# Autodesk Inventor assembly: COM
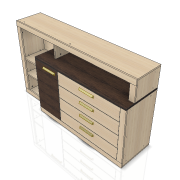
[picture p0: Inventor's stored thumbnail of the model, 180x180]
Saved by Autodesk Inventor 2024.3 (Build 283343000, 343)
## iProperties
Created: 2019-02-28
Document SubType Name: Assembly
Designer: SauliusD
Description: Commode
Part Number: COM
Author: SauliusD
## Documents named in this file (39)
- C:\W4INV 2024 Design\PROJECTS\Samples\Commode\COM.iam
- C:\W4INV 2024 Design\PROJECTS\Samples\Commode\COM_23.ipt
- C:\W4INV 2024 Design\PROJECTS\Samples\Commode\COM_10.ipt
- C:\W4INV 2024 Design\PROJECTS\Samples\Commode\COM_02.ipt
- C:\W4INV 2024 Design\PROJECTS\Samples\Commode\COM_16.ipt
- C:\W4INV 2024 Design\PROJECTS\Samples\Commode\COM_24.ipt
- C:\W4INV 2024 Design\PROJECTS\Samples\Commode\COM_11.ipt
- C:\W4INV 2024 Design\PROJECTS\Samples\Commode\COM_03.ipt
- C:\W4INV 2024 Design\PROJECTS\Samples\Commode\COM_17.ipt
- C:\W4INV 2024 Design\PROJECTS\Samples\Commode\COM_12.ipt
- C:\W4INV 2024 Design\PROJECTS\Samples\Commode\COM_25.ipt
- C:\W4INV 2024 Design\PROJECTS\Samples\Commode\COM_08.ipt
- C:\W4INV 2024 Design\PROJECTS\Samples\Commode\COM_04.ipt
- C:\W4INV 2024 Design\PROJECTS\Samples\Commode\COM_13.ipt
- C:\W4INV 2024 Design\PROJECTS\Samples\Commode\COM_05.ipt
- C:\W4INV 2024 Design\PROJECTS\Samples\Commode\COM_14.ipt
- C:\W4INV 2024 Design\PROJECTS\Samples\Commode\COM_18.ipt
- C:\W4INV 2024 Design\PROJECTS\Samples\Commode\COM_06.ipt
- C:\W4INV 2024 Design\PROJECTS\Samples\Commode\COM_07.ipt
- C:\W4INV 2024 Design\PROJECTS\Samples\Commode\COM_21.ipt
- C:\W4INV 2024 Design\PROJECTS\Samples\Commode\COM_20.ipt
- C:\W4INV 2024 Design\PROJECTS\Samples\Commode\COM_26.ipt
- C:\W4INV 2024 Design\PROJECTS\Samples\Commode\COM_19.ipt
- C:\W4INV 2024 Design\PROJECTS\Samples\Commode\COM_09.ipt
- C:\W4INV 2024 Design\PROJECTS\Samples\Commode\COM_15.ipt
- C:\W4INV 2024 Design\PROJECTS\Samples\Commode\SKL_COM_22.ipt
- C:\W4INV 2024 Design\PROJECTS\Samples\Commode\CommodePartial Pull Drawer 30 kg1\COM_01.iam
- C:\W4INV 2024 Design\_LIBRARY\Fixed joints\Minifix joint\MINIFIX D15 v2\Minifix D15 & Dowel L34 & Cap D15 PB T18 LH.ipt
- C:\W4INV 2024 Design\_LIBRARY\Holders\Shelf holder D5\Shelf support D5 L16 with hole covers.ipt
- C:\W4INV 2024 Design\_LIBRARY\Fixed joints\Dowel\DOWEL V2\Dowel 8x30 PB T=18.ipt
- C:\W4INV 2024 Design\_LIBRARY\Hinges\CONCEALED HINGE\Full Overlay Hinge Wood Screw Cup Wood Screw T18.iam
- C:\W4INV 2024 Design\_LIBRARY\Fixed joints\Minifix joint\MINIFIX D15 v2\Minifix D15 & Dowel L34 & Cap D15 PB T18 RH.ipt
- C:\W4INV 2024 Design\_LIBRARY\Fixed joints\Minifix joint\MINIFIX D15 v2\Minifix D15 & Dowel L34 & Cap D15 PB T18 BT.ipt
- C:\W4INV 2024 Design\PROJECTS\Samples\Commode\COM.iam Smart Hardware\ESTAMP Post 683110\ESTAMP Post 683110.iam
- C:\W4INV 2024 Design\PROJECTS\Samples\Commode\COM.iam Smart Hardware\ESTAMP Post 683111\ESTAMP Post 683111.iam
- C:\W4INV 2024 Design\LIBRARY\Fixed joints\Minifix joint\MINIFIX D15 v2.ipt
- C:\W4INV 2024 Design\LIBRARY\Holders\Shelf holder D5.ipt
- C:\W4INV 2024 Design\LIBRARY\Fixed joints\Dowel\DOWEL V2.ipt
- C:\W4INV 2024 Design\LIBRARY\Hinges\CONCEALED HINGE.iam
## Components (110 placed, 33 different names)
1. COM_23:1 — Axis Plane:1, Nestled Board Plane:1, Axis Plane:2, Nestled Board Plane:2, Axis Plane:3, Nestled Board Plane:3, Axis Plane:4, Nestled Board Plane:4, Axis Plane:5, Nestled Board Plane:5, Axis Plane:6, Nestled Board Plane:6, Axis Plane:7, Axis Plane:8, Axis Plane:9, Axis Plane:10, Axis Plane:11, Axis Plane:12, Axis Plane:29, Axis Plane:30, Axis Plane:31, Axis Plane:32, Axis Plane:33, Axis Plane:34, Axis Plane:35, Axis Plane:36, Pillar Board Side Plane :29, Pillar Board Side Plane :30, Pillar Board Side Plane :31, Axis Plane:69, Axis Plane:70
2. COM_10:1 — Pillar Board Side Plane :1, Pillar Board Side Plane :4, Pillar Board Side Plane :11, Pillar Board Side Plane :12, Side Board Plane:1, Side Board Plane:3, Side Board Plane:5, Side Board Plane:7, Pillar Board Side Plane :32, Pillar Board Side Plane :33, Pillar Board Side Plane :34
3. COM_02:1 — Nestled Board Plane:11, Nestled Board Plane:12, Pillar Board Side Plane :35, Pillar Board Side Plane :36, Pillar Board Side Plane :43, Pillar Board Side Plane :44
4. COM_16:1 — Pillar Board Side Plane :3, Pillar Board Side Plane :6, Pillar Board Side Plane :8, Pillar Board Side Plane :10
5. COM_24:1 — Nestled Board Plane:7, Nestled Board Plane:8, Nestled Board Plane:9, Nestled Board Plane:10, Axis Plane:13, Nestled Board Plane:13, Axis Plane:14, Axis Plane:15, Nestled Board Plane:15, Axis Plane:16, Axis Plane:17, Nestled Board Plane:17, Axis Plane:18, Axis Plane:19, Nestled Board Plane:19, Axis Plane:20, Axis Plane:21, Nestled Board Plane:21, Axis Plane:22, Axis Plane:23, Nestled Board Plane:23, Axis Plane:24, Axis Plane:25, Axis Plane:26, Axis Plane:27, Nestled Board Plane:27, Axis Plane:28, Nestled Board Plane:28, Axis Plane:37, Axis Plane:38, Axis Plane:39, Axis Plane:40, Axis Plane:41, Axis Plane:42, Axis Plane:43, Axis Plane:44, Nestled Board Plane:51, Nestled Board Plane:52
6. COM_11:1 — Pillar Board Side Plane :13, Pillar Board Side Plane :14, Pillar Board Side Plane :19, Pillar Board Side Plane :20, Side Board Plane:2, Side Board Plane:4, Side Board Plane:6, Side Board Plane:8, Side Board Plane:9, Side Board Plane:11, Side Board Plane:13, Side Board Plane:15, Cabinet Body Front  Edge Planar Face:1, Cabinet body Side Planar Face:1, Cabinet Body Front  Edge Planar Face:2, Cabinet body Side Planar Face:2, Nestled Board Plane:53, Nestled Board Plane:54
7. COM_03:1 — Nestled Board Plane:14, Nestled Board Plane:16, Nestled Board Plane:18, Nestled Board Plane:20, Nestled Board Plane:22, Nestled Board Plane:24, Nestled Board Plane:25, Nestled Board Plane:26, Pillar Board Side Plane :37, Pillar Board Side Plane :38, Pillar Board Side Plane :39
8. COM_17:1 — Pillar Board Side Plane :25, Pillar Board Side Plane :26, Pillar Board Side Plane :27, Pillar Board Side Plane :28, Pillar Board Side Plane :40, Pillar Board Side Plane :41, Pillar Board Side Plane :42
9. COM_12:1 — Pillar Board Side Plane :15, Pillar Board Side Plane :16, Pillar Board Side Plane :21, Pillar Board Side Plane :22, Side Board Plane:10, Side Board Plane:12, Side Board Plane:14, Side Board Plane:16
10. COM_25:1 — Axis Plane:45, Nestled Board Plane:29, Axis Plane:46, Nestled Board Plane:30, Axis Plane:47, Nestled Board Plane:31, Nestled Board Plane:43, Nestled Board Plane:44, Nestled Board Plane:45, Nestled Board Plane:46, Nestled Board Plane:49, Nestled Board Plane:50
11. COM_08:1 — Axis Plane:48, Nestled Board Plane:32, Axis Plane:49, Nestled Board Plane:33, Axis Plane:50, Nestled Board Plane:34, Axis Plane:59, Pillar Board Plane:1, Axis Plane:60, Pillar Board Plane:2, Pillar Board Plane:3, Pillar Board Plane:4, Axis Plane:63, Pillar Board Plane:5, Axis Plane:64, Pillar Board Plane:6
12. COM_04:1 — Axis Plane:51, Nestled Board Plane:35, Axis Plane:52, Nestled Board Plane:36, Nestled Board Plane:47, Nestled Board Plane:48
13. COM_13:1 — Axis Plane:61, Axis Plane:62, Axis Plane:65, Pillar Board Plane:7, Axis Plane:66, Pillar Board Plane:8, Axis Plane:67, Pillar Board Plane:9, Axis Plane:68, Pillar Board Plane:10
14. COM_05:1 — Axis Plane:53, Nestled Board Plane:37, Axis Plane:54, Nestled Board Plane:38, Axis Plane:55, Nestled Board Plane:39
15. COM_14:1 — Axis Plane:56, Nestled Board Plane:40, Axis Plane:57, Nestled Board Plane:41, Axis Plane:58, Nestled Board Plane:42
16. COM_18:1 — Pillar Board Side Plane :17, Pillar Board Side Plane :18, Pillar Board Side Plane :23, Pillar Board Side Plane :24
17. COM_06:1 — Flush:46, Flush:47
18. COM_21:1 — Top of drawer Box:1, Front of drawer Box:1, Right of drawer Box:1
19. COM_26:1 — Pillar Board Side Plane :2, Pillar Board Side Plane :5, Pillar Board Side Plane :7, Pillar Board Side Plane :9
20. COM_09:1
21. COM_15:1
22. Minifix D15 & Dowel L34 & Cap D15 PB T18 LH:2 — Axis Plane:1, Pillar Board Side Plane :1, Nestled Board Plane:1
23. Minifix D15 & Dowel L34 & Cap D15 PB T18 LH:3 — Axis Plane:2, Pillar Board Side Plane :2, Nestled Board Plane:2
24. Minifix D15 & Dowel L34 & Cap D15 PB T18 RH:4 — Axis Plane:3, Pillar Board Side Plane :3, Nestled Board Plane:3
25. Minifix D15 & Dowel L34 & Cap D15 PB T18 RH:5 — Axis Plane:4, Pillar Board Side Plane :4, Nestled Board Plane:4
26. Minifix D15 & Dowel L34 & Cap D15 PB T18 RH:6 — Axis Plane:5, Pillar Board Side Plane :5, Nestled Board Plane:5
27. Minifix D15 & Dowel L34 & Cap D15 PB T18 LH:7 — Axis Plane:6, Pillar Board Side Plane :6, Nestled Board Plane:6
28. Minifix D15 & Dowel L34 & Cap D15 PB T18 LH:8 — Axis Plane:7, Pillar Board Side Plane :7, Nestled Board Plane:7
29. Minifix D15 & Dowel L34 & Cap D15 PB T18 RH:9 — Axis Plane:8, Pillar Board Side Plane :8, Nestled Board Plane:8
30. Minifix D15 & Dowel L34 & Cap D15 PB T18 RH:10 — Axis Plane:9, Pillar Board Side Plane :9, Nestled Board Plane:9
31. Minifix D15 & Dowel L34 & Cap D15 PB T18 LH:11 — Axis Plane:10, Pillar Board Side Plane :10, Nestled Board Plane:10
32. Minifix D15 & Dowel L34 & Cap D15 PB T18 RH:12 — Axis Plane:11, Nestled Board Plane:11, Pillar Board Side Plane :11
33. Minifix D15 & Dowel L34 & Cap D15 PB T18 LH:13 — Axis Plane:12, Nestled Board Plane:12, Pillar Board Side Plane :12
34. Minifix D15 & Dowel L34 & Cap D15 PB T18 LH:14 — Axis Plane:13, Pillar Board Side Plane :13, Nestled Board Plane:13
35. Minifix D15 & Dowel L34 & Cap D15 PB T18 RH:15 — Axis Plane:14, Pillar Board Side Plane :14, Nestled Board Plane:14
36. Minifix D15 & Dowel L34 & Cap D15 PB T18 LH:16 — Axis Plane:15, Pillar Board Side Plane :15, Nestled Board Plane:15
37. Minifix D15 & Dowel L34 & Cap D15 PB T18 LH:17 — Axis Plane:16, Pillar Board Side Plane :16, Nestled Board Plane:16
38. Minifix D15 & Dowel L34 & Cap D15 PB T18 RH:18 — Axis Plane:17, Pillar Board Side Plane :17, Nestled Board Plane:17
39. Minifix D15 & Dowel L34 & Cap D15 PB T18 LH:19 — Axis Plane:18, Pillar Board Side Plane :18, Nestled Board Plane:18
40. Minifix D15 & Dowel L34 & Cap D15 PB T18 LH:20 — Axis Plane:19, Pillar Board Side Plane :19, Nestled Board Plane:19
41. Minifix D15 & Dowel L34 & Cap D15 PB T18 LH:21 — Axis Plane:20, Pillar Board Side Plane :20, Nestled Board Plane:20
42. Minifix D15 & Dowel L34 & Cap D15 PB T18 RH:22 — Axis Plane:21, Pillar Board Side Plane :21, Nestled Board Plane:21
43. Minifix D15 & Dowel L34 & Cap D15 PB T18 LH:23 — Axis Plane:22, Pillar Board Side Plane :22, Nestled Board Plane:22
44. Minifix D15 & Dowel L34 & Cap D15 PB T18 LH:24 — Axis Plane:23, Pillar Board Side Plane :23, Nestled Board Plane:23
45. Minifix D15 & Dowel L34 & Cap D15 PB T18 RH:25 — Axis Plane:24, Pillar Board Side Plane :24, Nestled Board Plane:24
46. Minifix D15 & Dowel L34 & Cap D15 PB T18 LH:26 — Axis Plane:25, Nestled Board Plane:25, Pillar Board Side Plane :25
47. Minifix D15 & Dowel L34 & Cap D15 PB T18 RH:27 — Axis Plane:26, Nestled Board Plane:26, Pillar Board Side Plane :26
48. Minifix D15 & Dowel L34 & Cap D15 PB T18 LH:28 — Axis Plane:27, Nestled Board Plane:27, Pillar Board Side Plane :27
49. Minifix D15 & Dowel L34 & Cap D15 PB T18 LH:29 — Axis Plane:28, Nestled Board Plane:28, Pillar Board Side Plane :28
50. Shelf support D5 L16 with hole covers:1 — Axis Plane:29, Shelf Pottom Plane:1, Side Board Plane:1
51. Shelf support D5 L16 with hole covers:2 — Axis Plane:30, Shelf Pottom Plane:2, Side Board Plane:2
52. Shelf support D5 L16 with hole covers:3 — Axis Plane:31, Shelf Pottom Plane:3, Side Board Plane:3
53. Shelf support D5 L16 with hole covers:4 — Axis Plane:32, Shelf Pottom Plane:4, Side Board Plane:4
54. Shelf support D5 L16 with hole covers:5 — Axis Plane:33, Shelf Pottom Plane:5, Side Board Plane:5
55. Shelf support D5 L16 with hole covers:6 — Axis Plane:34, Shelf Pottom Plane:6, Side Board Plane:6
56. Shelf support D5 L16 with hole covers:7 — Axis Plane:35, Shelf Pottom Plane:7, Side Board Plane:7
57. Shelf support D5 L16 with hole covers:8 — Axis Plane:36, Shelf Pottom Plane:8, Side Board Plane:8
58. Shelf support D5 L16 with hole covers:9 — Axis Plane:37, Shelf Pottom Plane:9, Side Board Plane:9
59. Shelf support D5 L16 with hole covers:10 — Axis Plane:38, Shelf Pottom Plane:10, Side Board Plane:10
60. Shelf support D5 L16 with hole covers:11 — Axis Plane:39, Shelf Pottom Plane:11, Side Board Plane:11
61. Shelf support D5 L16 with hole covers:12 — Axis Plane:40, Shelf Pottom Plane:12, Side Board Plane:12
62. Shelf support D5 L16 with hole covers:13 — Axis Plane:41, Shelf Pottom Plane:13, Side Board Plane:13
63. Shelf support D5 L16 with hole covers:14 — Axis Plane:42, Shelf Pottom Plane:14, Side Board Plane:14
64. Shelf support D5 L16 with hole covers:15 — Axis Plane:43, Shelf Pottom Plane:15, Side Board Plane:15
65. Shelf support D5 L16 with hole covers:16 — Axis Plane:44, Shelf Pottom Plane:16, Side Board Plane:16
66. Minifix D15 & Dowel L34 & Cap D15 PB T18 LH:30 — Axis Plane:45, Nestled Board Plane:29, Pillar Board Side Plane :29
67. Minifix D15 & Dowel L34 & Cap D15 PB T18 BT:31 — Axis Plane:46, Nestled Board Plane:30, Pillar Board Side Plane :30
68. Minifix D15 & Dowel L34 & Cap D15 PB T18 LH:32 — Axis Plane:47, Nestled Board Plane:31, Pillar Board Side Plane :31
69. Minifix D15 & Dowel L34 & Cap D15 PB T18 RH:33 — Axis Plane:48, Nestled Board Plane:32, Pillar Board Side Plane :32
70. Minifix D15 & Dowel L34 & Cap D15 PB T18 BT:34 — Axis Plane:49, Nestled Board Plane:33, Pillar Board Side Plane :33
71. Minifix D15 & Dowel L34 & Cap D15 PB T18 LH:35 — Axis Plane:50, Nestled Board Plane:34, Pillar Board Side Plane :34
72. Minifix D15 & Dowel L34 & Cap D15 PB T18 RH:36 — Axis Plane:51, Nestled Board Plane:35, Pillar Board Side Plane :35
73. Minifix D15 & Dowel L34 & Cap D15 PB T18 LH:37 — Axis Plane:52, Nestled Board Plane:36, Pillar Board Side Plane :36
74. Minifix D15 & Dowel L34 & Cap D15 PB T18 RH:38 — Axis Plane:53, Nestled Board Plane:37, Pillar Board Side Plane :37
75. Minifix D15 & Dowel L34 & Cap D15 PB T18 BT:39 — Axis Plane:54, Nestled Board Plane:38, Pillar Board Side Plane :38
76. Minifix D15 & Dowel L34 & Cap D15 PB T18 LH:40 — Axis Plane:55, Nestled Board Plane:39, Pillar Board Side Plane :39
77. Minifix D15 & Dowel L34 & Cap D15 PB T18 LH:41 — Axis Plane:56, Nestled Board Plane:40, Pillar Board Side Plane :40
78. Minifix D15 & Dowel L34 & Cap D15 PB T18 BT:42 — Axis Plane:57, Nestled Board Plane:41, Pillar Board Side Plane :41
79. Minifix D15 & Dowel L34 & Cap D15 PB T18 RH:43 — Axis Plane:58, Nestled Board Plane:42, Pillar Board Side Plane :42
80. Dowel 8x30 PB T=18:1 — Axis Plane:59, Nestled Board Plane:43, Pillar Board Plane:1
81. Dowel 8x30 PB T=18:2 — Axis Plane:60, Nestled Board Plane:44, Pillar Board Plane:2
82. Dowel 8x30 PB T=18:3 — Axis Plane:61, Nestled Board Plane:45, Pillar Board Plane:3
83. Dowel 8x30 PB T=18:4 — Axis Plane:62, Nestled Board Plane:46, Pillar Board Plane:4
84. Dowel 8x30 PB T=18:5 — Axis Plane:63, Nestled Board Plane:47, Pillar Board Plane:5
85. Dowel 8x30 PB T=18:6 — Axis Plane:64, Nestled Board Plane:48, Pillar Board Plane:6
86. Dowel 8x30 PB T=18:7 — Axis Plane:65, Nestled Board Plane:49, Pillar Board Plane:7
87. Dowel 8x30 PB T=18:8 — Axis Plane:66, Nestled Board Plane:50, Pillar Board Plane:8
88. Dowel 8x30 PB T=18:9 — Axis Plane:67, Nestled Board Plane:51, Pillar Board Plane:9
89. Dowel 8x30 PB T=18:10 — Axis Plane:68, Nestled Board Plane:52, Pillar Board Plane:10
90. Full Overlay Hinge Wood Screw Cup Wood Screw T18:1 [sub-assembly] — Hinge Center Axis Plane:1, Cabinet Body Front  Edge Planar Face:1, Cabinet body Side Planar Face:1
91. Full Overlay Hinge Wood Screw Cup Wood Screw T18:2 [sub-assembly] — Hinge Center Axis Plane:2, Cabinet Body Front  Edge Planar Face:2, Cabinet body Side Planar Face:2
92. Minifix D15 & Dowel L34 & Cap D15 PB T18 LH:45 — Axis Plane:69, Nestled Board Plane:53, Pillar Board Side Plane :43
93. Minifix D15 & Dowel L34 & Cap D15 PB T18 RH:46 — Axis Plane:70, Nestled Board Plane:54, Pillar Board Side Plane :44
94. ESTAMP Post 683111:1 [sub-assembly]
95. COM_07:1
96. ESTAMP Post 683110:1 [sub-assembly]
97. COM_07:2
98. ESTAMP Post 683110:2 [sub-assembly]
99. COM_07:3
100. ESTAMP Post 683110:3 [sub-assembly]
101. COM_07:4
102. ESTAMP Post 683110:4 [sub-assembly]
103. COM_20:1 — Shelf Pottom Plane:1, Shelf Pottom Plane:2, Shelf Pottom Plane:5, Shelf Pottom Plane:6
104. COM_20:2 — Shelf Pottom Plane:3, Shelf Pottom Plane:4, Shelf Pottom Plane:7, Shelf Pottom Plane:8
105. COM_19:1 — Shelf Pottom Plane:9, Shelf Pottom Plane:10, Shelf Pottom Plane:13, Shelf Pottom Plane:14
106. COM_19:2 — Shelf Pottom Plane:11, Shelf Pottom Plane:12, Shelf Pottom Plane:15, Shelf Pottom Plane:16
107. COM_01:1 [sub-assembly] — Top of drawer Box:1, Front of drawer Box:1, Right of drawer Box:1
108. COM_01:2 [sub-assembly]
109. COM_01:3 [sub-assembly]
110. COM_01:4 [sub-assembly]
## Component patterns: (4 elements, first: COM_07:1 + ESTAMP Post 683110:1), (2 elements, first: COM_20:1), (2 elements, first: COM_19:1), (4 elements, first: COM_01:1)
## Relationships (221: Mate 170, Flush 51)
- Top of drawer Box:1 [Flush]: COM_21:1 ↔ COM_01:1
- Front of drawer Box:1 [Flush]: COM_21:1 ↔ COM_01:1
- Right of drawer Box:1 [Flush]: COM_21:1 ↔ COM_01:1
- Axis Plane:1 [Mate]: COM_23:1 ↔ Minifix D15 & Dowel L34 & Cap D15 PB T18 LH:2
- Pillar Board Side Plane :1 [Flush] (18 mm): COM_10:1 ↔ Minifix D15 & Dowel L34 & Cap D15 PB T18 LH:2
- Nestled Board Plane:1 [Mate]: COM_23:1 ↔ Minifix D15 & Dowel L34 & Cap D15 PB T18 LH:2
- Axis Plane:2 [Mate]: COM_23:1 ↔ Minifix D15 & Dowel L34 & Cap D15 PB T18 LH:3
- Pillar Board Side Plane :2 [Flush] (18 mm): COM_26:1 ↔ Minifix D15 & Dowel L34 & Cap D15 PB T18 LH:3
- Nestled Board Plane:2 [Mate]: COM_23:1 ↔ Minifix D15 & Dowel L34 & Cap D15 PB T18 LH:3
- Axis Plane:3 [Mate]: COM_23:1 ↔ Minifix D15 & Dowel L34 & Cap D15 PB T18 RH:4
- Pillar Board Side Plane :3 [Flush] (18 mm): COM_16:1 ↔ Minifix D15 & Dowel L34 & Cap D15 PB T18 RH:4
- Nestled Board Plane:3 [Mate]: COM_23:1 ↔ Minifix D15 & Dowel L34 & Cap D15 PB T18 RH:4
- Axis Plane:4 [Mate]: COM_23:1 ↔ Minifix D15 & Dowel L34 & Cap D15 PB T18 RH:5
- Pillar Board Side Plane :4 [Flush] (18 mm): COM_10:1 ↔ Minifix D15 & Dowel L34 & Cap D15 PB T18 RH:5
- Nestled Board Plane:4 [Mate]: COM_23:1 ↔ Minifix D15 & Dowel L34 & Cap D15 PB T18 RH:5
- Axis Plane:5 [Mate]: COM_23:1 ↔ Minifix D15 & Dowel L34 & Cap D15 PB T18 RH:6
- Pillar Board Side Plane :5 [Flush] (18 mm): COM_26:1 ↔ Minifix D15 & Dowel L34 & Cap D15 PB T18 RH:6
- Nestled Board Plane:5 [Mate]: COM_23:1 ↔ Minifix D15 & Dowel L34 & Cap D15 PB T18 RH:6
- Axis Plane:6 [Mate]: COM_23:1 ↔ Minifix D15 & Dowel L34 & Cap D15 PB T18 LH:7
- Pillar Board Side Plane :6 [Flush] (18 mm): COM_16:1 ↔ Minifix D15 & Dowel L34 & Cap D15 PB T18 LH:7
- Nestled Board Plane:6 [Mate]: COM_23:1 ↔ Minifix D15 & Dowel L34 & Cap D15 PB T18 LH:7
- Axis Plane:7 [Mate]: COM_23:1 ↔ Minifix D15 & Dowel L34 & Cap D15 PB T18 LH:8
- Pillar Board Side Plane :7 [Flush] (18 mm): COM_26:1 ↔ Minifix D15 & Dowel L34 & Cap D15 PB T18 LH:8
- Nestled Board Plane:7 [Mate]: COM_24:1 ↔ Minifix D15 & Dowel L34 & Cap D15 PB T18 LH:8
- Axis Plane:8 [Mate]: COM_23:1 ↔ Minifix D15 & Dowel L34 & Cap D15 PB T18 RH:9
- Pillar Board Side Plane :8 [Flush] (18 mm): COM_16:1 ↔ Minifix D15 & Dowel L34 & Cap D15 PB T18 RH:9
- Nestled Board Plane:8 [Mate]: COM_24:1 ↔ Minifix D15 & Dowel L34 & Cap D15 PB T18 RH:9
- Axis Plane:9 [Mate]: COM_23:1 ↔ Minifix D15 & Dowel L34 & Cap D15 PB T18 RH:10
- Pillar Board Side Plane :9 [Flush] (18 mm): COM_26:1 ↔ Minifix D15 & Dowel L34 & Cap D15 PB T18 RH:10
- Nestled Board Plane:9 [Mate]: COM_24:1 ↔ Minifix D15 & Dowel L34 & Cap D15 PB T18 RH:10
- Axis Plane:10 [Mate]: COM_23:1 ↔ Minifix D15 & Dowel L34 & Cap D15 PB T18 LH:11
- Pillar Board Side Plane :10 [Flush] (18 mm): COM_16:1 ↔ Minifix D15 & Dowel L34 & Cap D15 PB T18 LH:11
- Nestled Board Plane:10 [Mate]: COM_24:1 ↔ Minifix D15 & Dowel L34 & Cap D15 PB T18 LH:11
- Axis Plane:11 [Mate]: COM_23:1 ↔ Minifix D15 & Dowel L34 & Cap D15 PB T18 RH:12
- Nestled Board Plane:11 [Mate]: COM_02:1 ↔ Minifix D15 & Dowel L34 & Cap D15 PB T18 RH:12
- Pillar Board Side Plane :11 [Flush] (18 mm): COM_10:1 ↔ Minifix D15 & Dowel L34 & Cap D15 PB T18 RH:12
- Axis Plane:12 [Mate]: COM_23:1 ↔ Minifix D15 & Dowel L34 & Cap D15 PB T18 LH:13
- Nestled Board Plane:12 [Mate]: COM_02:1 ↔ Minifix D15 & Dowel L34 & Cap D15 PB T18 LH:13
- Pillar Board Side Plane :12 [Flush] (18 mm): COM_10:1 ↔ Minifix D15 & Dowel L34 & Cap D15 PB T18 LH:13
- Axis Plane:13 [Mate]: COM_24:1 ↔ Minifix D15 & Dowel L34 & Cap D15 PB T18 LH:14
- Pillar Board Side Plane :13 [Flush] (18 mm): COM_11:1 ↔ Minifix D15 & Dowel L34 & Cap D15 PB T18 LH:14
- Nestled Board Plane:13 [Mate]: COM_24:1 ↔ Minifix D15 & Dowel L34 & Cap D15 PB T18 LH:14
- Axis Plane:14 [Mate]: COM_24:1 ↔ Minifix D15 & Dowel L34 & Cap D15 PB T18 RH:15
- Pillar Board Side Plane :14 [Flush] (18 mm): COM_11:1 ↔ Minifix D15 & Dowel L34 & Cap D15 PB T18 RH:15
- Nestled Board Plane:14 [Mate]: COM_03:1 ↔ Minifix D15 & Dowel L34 & Cap D15 PB T18 RH:15
- Axis Plane:15 [Mate]: COM_24:1 ↔ Minifix D15 & Dowel L34 & Cap D15 PB T18 LH:16
- Pillar Board Side Plane :15 [Flush] (18 mm): COM_12:1 ↔ Minifix D15 & Dowel L34 & Cap D15 PB T18 LH:16
- Nestled Board Plane:15 [Mate]: COM_24:1 ↔ Minifix D15 & Dowel L34 & Cap D15 PB T18 LH:16
- Axis Plane:16 [Mate]: COM_24:1 ↔ Minifix D15 & Dowel L34 & Cap D15 PB T18 LH:17
- Pillar Board Side Plane :16 [Flush] (18 mm): COM_12:1 ↔ Minifix D15 & Dowel L34 & Cap D15 PB T18 LH:17
- Nestled Board Plane:16 [Mate]: COM_03:1 ↔ Minifix D15 & Dowel L34 & Cap D15 PB T18 LH:17
- Axis Plane:17 [Mate]: COM_24:1 ↔ Minifix D15 & Dowel L34 & Cap D15 PB T18 RH:18
- Pillar Board Side Plane :17 [Flush] (18 mm): COM_18:1 ↔ Minifix D15 & Dowel L34 & Cap D15 PB T18 RH:18
- Nestled Board Plane:17 [Mate]: COM_24:1 ↔ Minifix D15 & Dowel L34 & Cap D15 PB T18 RH:18
- Axis Plane:18 [Mate]: COM_24:1 ↔ Minifix D15 & Dowel L34 & Cap D15 PB T18 LH:19
- Pillar Board Side Plane :18 [Flush] (18 mm): COM_18:1 ↔ Minifix D15 & Dowel L34 & Cap D15 PB T18 LH:19
- Nestled Board Plane:18 [Mate]: COM_03:1 ↔ Minifix D15 & Dowel L34 & Cap D15 PB T18 LH:19
- Axis Plane:19 [Mate]: COM_24:1 ↔ Minifix D15 & Dowel L34 & Cap D15 PB T18 LH:20
- Pillar Board Side Plane :19 [Flush] (18 mm): COM_11:1 ↔ Minifix D15 & Dowel L34 & Cap D15 PB T18 LH:20
- Nestled Board Plane:19 [Mate]: COM_24:1 ↔ Minifix D15 & Dowel L34 & Cap D15 PB T18 LH:20
- Axis Plane:20 [Mate]: COM_24:1 ↔ Minifix D15 & Dowel L34 & Cap D15 PB T18 LH:21
- Pillar Board Side Plane :20 [Flush] (18 mm): COM_11:1 ↔ Minifix D15 & Dowel L34 & Cap D15 PB T18 LH:21
- Nestled Board Plane:20 [Mate]: COM_03:1 ↔ Minifix D15 & Dowel L34 & Cap D15 PB T18 LH:21
- Axis Plane:21 [Mate]: COM_24:1 ↔ Minifix D15 & Dowel L34 & Cap D15 PB T18 RH:22
- Pillar Board Side Plane :21 [Flush] (18 mm): COM_12:1 ↔ Minifix D15 & Dowel L34 & Cap D15 PB T18 RH:22
- Nestled Board Plane:21 [Mate]: COM_24:1 ↔ Minifix D15 & Dowel L34 & Cap D15 PB T18 RH:22
- Axis Plane:22 [Mate]: COM_24:1 ↔ Minifix D15 & Dowel L34 & Cap D15 PB T18 LH:23
- Pillar Board Side Plane :22 [Flush] (18 mm): COM_12:1 ↔ Minifix D15 & Dowel L34 & Cap D15 PB T18 LH:23
- Nestled Board Plane:22 [Mate]: COM_03:1 ↔ Minifix D15 & Dowel L34 & Cap D15 PB T18 LH:23
- Axis Plane:23 [Mate]: COM_24:1 ↔ Minifix D15 & Dowel L34 & Cap D15 PB T18 LH:24
- Pillar Board Side Plane :23 [Flush] (18 mm): COM_18:1 ↔ Minifix D15 & Dowel L34 & Cap D15 PB T18 LH:24
- Nestled Board Plane:23 [Mate]: COM_24:1 ↔ Minifix D15 & Dowel L34 & Cap D15 PB T18 LH:24
- Axis Plane:24 [Mate]: COM_24:1 ↔ Minifix D15 & Dowel L34 & Cap D15 PB T18 RH:25
- Pillar Board Side Plane :24 [Flush] (18 mm): COM_18:1 ↔ Minifix D15 & Dowel L34 & Cap D15 PB T18 RH:25
- Nestled Board Plane:24 [Mate]: COM_03:1 ↔ Minifix D15 & Dowel L34 & Cap D15 PB T18 RH:25
- Axis Plane:25 [Mate]: COM_24:1 ↔ Minifix D15 & Dowel L34 & Cap D15 PB T18 LH:26
- Nestled Board Plane:25 [Mate]: COM_03:1 ↔ Minifix D15 & Dowel L34 & Cap D15 PB T18 LH:26
- Pillar Board Side Plane :25 [Flush] (18 mm): COM_17:1 ↔ Minifix D15 & Dowel L34 & Cap D15 PB T18 LH:26
- Axis Plane:26 [Mate]: COM_24:1 ↔ Minifix D15 & Dowel L34 & Cap D15 PB T18 RH:27
- Nestled Board Plane:26 [Mate]: COM_03:1 ↔ Minifix D15 & Dowel L34 & Cap D15 PB T18 RH:27
- Pillar Board Side Plane :26 [Flush] (18 mm): COM_17:1 ↔ Minifix D15 & Dowel L34 & Cap D15 PB T18 RH:27
- Axis Plane:27 [Mate]: COM_24:1 ↔ Minifix D15 & Dowel L34 & Cap D15 PB T18 LH:28
- Nestled Board Plane:27 [Mate]: COM_24:1 ↔ Minifix D15 & Dowel L34 & Cap D15 PB T18 LH:28
- Pillar Board Side Plane :27 [Flush] (18 mm): COM_17:1 ↔ Minifix D15 & Dowel L34 & Cap D15 PB T18 LH:28
- Axis Plane:28 [Mate]: COM_24:1 ↔ Minifix D15 & Dowel L34 & Cap D15 PB T18 LH:29
- Nestled Board Plane:28 [Mate]: COM_24:1 ↔ Minifix D15 & Dowel L34 & Cap D15 PB T18 LH:29
- Pillar Board Side Plane :28 [Flush] (18 mm): COM_17:1 ↔ Minifix D15 & Dowel L34 & Cap D15 PB T18 LH:29
- Axis Plane:29 [Mate]: COM_23:1 ↔ Shelf support D5 L16 with hole covers:1
- Shelf Pottom Plane:1 [Mate] (2.5 mm): Shelf support D5 L16 with hole covers:1 ↔ COM_20:1
- Side Board Plane:1 [Mate]: COM_10:1 ↔ Shelf support D5 L16 with hole covers:1
- Axis Plane:30 [Mate]: COM_23:1 ↔ Shelf support D5 L16 with hole covers:2
- Shelf Pottom Plane:2 [Mate] (2.5 mm): Shelf support D5 L16 with hole covers:2 ↔ COM_20:1
- Side Board Plane:2 [Mate]: COM_11:1 ↔ Shelf support D5 L16 with hole covers:2
- Axis Plane:31 [Mate]: COM_23:1 ↔ Shelf support D5 L16 with hole covers:3
- Shelf Pottom Plane:3 [Mate] (2.5 mm): Shelf support D5 L16 with hole covers:3 ↔ COM_20:2
- Side Board Plane:3 [Mate]: COM_10:1 ↔ Shelf support D5 L16 with hole covers:3
- Axis Plane:32 [Mate]: COM_23:1 ↔ Shelf support D5 L16 with hole covers:4
- Shelf Pottom Plane:4 [Mate] (2.5 mm): Shelf support D5 L16 with hole covers:4 ↔ COM_20:2
- Side Board Plane:4 [Mate]: COM_11:1 ↔ Shelf support D5 L16 with hole covers:4
- Axis Plane:33 [Mate]: COM_23:1 ↔ Shelf support D5 L16 with hole covers:5
- Shelf Pottom Plane:5 [Mate] (2.5 mm): Shelf support D5 L16 with hole covers:5 ↔ COM_20:1
- Side Board Plane:5 [Mate]: COM_10:1 ↔ Shelf support D5 L16 with hole covers:5
- Axis Plane:34 [Mate]: COM_23:1 ↔ Shelf support D5 L16 with hole covers:6
- Shelf Pottom Plane:6 [Mate] (2.5 mm): Shelf support D5 L16 with hole covers:6 ↔ COM_20:1
- Side Board Plane:6 [Mate]: COM_11:1 ↔ Shelf support D5 L16 with hole covers:6
- Axis Plane:35 [Mate]: COM_23:1 ↔ Shelf support D5 L16 with hole covers:7
- Shelf Pottom Plane:7 [Mate] (2.5 mm): Shelf support D5 L16 with hole covers:7 ↔ COM_20:2
- Side Board Plane:7 [Mate]: COM_10:1 ↔ Shelf support D5 L16 with hole covers:7
- Axis Plane:36 [Mate]: COM_23:1 ↔ Shelf support D5 L16 with hole covers:8
- Shelf Pottom Plane:8 [Mate] (2.5 mm): Shelf support D5 L16 with hole covers:8 ↔ COM_20:2
- Side Board Plane:8 [Mate]: COM_11:1 ↔ Shelf support D5 L16 with hole covers:8
- Axis Plane:37 [Mate]: COM_24:1 ↔ Shelf support D5 L16 with hole covers:9
- Shelf Pottom Plane:9 [Mate] (2.5 mm): Shelf support D5 L16 with hole covers:9 ↔ COM_19:1
- Side Board Plane:9 [Mate]: COM_11:1 ↔ Shelf support D5 L16 with hole covers:9
- Axis Plane:38 [Mate]: COM_24:1 ↔ Shelf support D5 L16 with hole covers:10
- Shelf Pottom Plane:10 [Mate] (2.5 mm): Shelf support D5 L16 with hole covers:10 ↔ COM_19:1
- Side Board Plane:10 [Mate]: COM_12:1 ↔ Shelf support D5 L16 with hole covers:10
- Axis Plane:39 [Mate]: COM_24:1 ↔ Shelf support D5 L16 with hole covers:11
- Shelf Pottom Plane:11 [Mate] (2.5 mm): Shelf support D5 L16 with hole covers:11 ↔ COM_19:2
- Side Board Plane:11 [Mate]: COM_11:1 ↔ Shelf support D5 L16 with hole covers:11
- Axis Plane:40 [Mate]: COM_24:1 ↔ Shelf support D5 L16 with hole covers:12
- Shelf Pottom Plane:12 [Mate] (2.5 mm): Shelf support D5 L16 with hole covers:12 ↔ COM_19:2
- Side Board Plane:12 [Mate]: COM_12:1 ↔ Shelf support D5 L16 with hole covers:12
- Axis Plane:41 [Mate]: COM_24:1 ↔ Shelf support D5 L16 with hole covers:13
- Shelf Pottom Plane:13 [Mate] (2.5 mm): Shelf support D5 L16 with hole covers:13 ↔ COM_19:1
- Side Board Plane:13 [Mate]: COM_11:1 ↔ Shelf support D5 L16 with hole covers:13
- Axis Plane:42 [Mate]: COM_24:1 ↔ Shelf support D5 L16 with hole covers:14
- Shelf Pottom Plane:14 [Mate] (2.5 mm): Shelf support D5 L16 with hole covers:14 ↔ COM_19:1
- Side Board Plane:14 [Mate]: COM_12:1 ↔ Shelf support D5 L16 with hole covers:14
- Axis Plane:43 [Mate]: COM_24:1 ↔ Shelf support D5 L16 with hole covers:15
- Shelf Pottom Plane:15 [Mate] (2.5 mm): Shelf support D5 L16 with hole covers:15 ↔ COM_19:2
- Side Board Plane:15 [Mate]: COM_11:1 ↔ Shelf support D5 L16 with hole covers:15
- Axis Plane:44 [Mate]: COM_24:1 ↔ Shelf support D5 L16 with hole covers:16
- Shelf Pottom Plane:16 [Mate] (2.5 mm): Shelf support D5 L16 with hole covers:16 ↔ COM_19:2
- Side Board Plane:16 [Mate]: COM_12:1 ↔ Shelf support D5 L16 with hole covers:16
- Axis Plane:45 [Mate]: COM_25:1 ↔ Minifix D15 & Dowel L34 & Cap D15 PB T18 LH:30
- Nestled Board Plane:29 [Mate]: COM_25:1 ↔ Minifix D15 & Dowel L34 & Cap D15 PB T18 LH:30
- Pillar Board Side Plane :29 [Flush] (18 mm): COM_23:1 ↔ Minifix D15 & Dowel L34 & Cap D15 PB T18 LH:30
- Axis Plane:46 [Mate]: COM_25:1 ↔ Minifix D15 & Dowel L34 & Cap D15 PB T18 BT:31
- Nestled Board Plane:30 [Mate]: COM_25:1 ↔ Minifix D15 & Dowel L34 & Cap D15 PB T18 BT:31
- Pillar Board Side Plane :30 [Flush] (18 mm): COM_23:1 ↔ Minifix D15 & Dowel L34 & Cap D15 PB T18 BT:31
- Axis Plane:47 [Mate]: COM_25:1 ↔ Minifix D15 & Dowel L34 & Cap D15 PB T18 LH:32
- Nestled Board Plane:31 [Mate]: COM_25:1 ↔ Minifix D15 & Dowel L34 & Cap D15 PB T18 LH:32
- Pillar Board Side Plane :31 [Flush] (18 mm): COM_23:1 ↔ Minifix D15 & Dowel L34 & Cap D15 PB T18 LH:32
- Axis Plane:48 [Mate]: COM_08:1 ↔ Minifix D15 & Dowel L34 & Cap D15 PB T18 RH:33
- Nestled Board Plane:32 [Mate]: COM_08:1 ↔ Minifix D15 & Dowel L34 & Cap D15 PB T18 RH:33
- Pillar Board Side Plane :32 [Flush] (18 mm): COM_10:1 ↔ Minifix D15 & Dowel L34 & Cap D15 PB T18 RH:33
- Axis Plane:49 [Mate]: COM_08:1 ↔ Minifix D15 & Dowel L34 & Cap D15 PB T18 BT:34
- Nestled Board Plane:33 [Mate]: COM_08:1 ↔ Minifix D15 & Dowel L34 & Cap D15 PB T18 BT:34
- Pillar Board Side Plane :33 [Flush] (18 mm): COM_10:1 ↔ Minifix D15 & Dowel L34 & Cap D15 PB T18 BT:34
- Axis Plane:50 [Mate]: COM_08:1 ↔ Minifix D15 & Dowel L34 & Cap D15 PB T18 LH:35
- Nestled Board Plane:34 [Mate]: COM_08:1 ↔ Minifix D15 & Dowel L34 & Cap D15 PB T18 LH:35
- Pillar Board Side Plane :34 [Flush] (18 mm): COM_10:1 ↔ Minifix D15 & Dowel L34 & Cap D15 PB T18 LH:35
- Axis Plane:51 [Mate]: COM_04:1 ↔ Minifix D15 & Dowel L34 & Cap D15 PB T18 RH:36
- Nestled Board Plane:35 [Mate]: COM_04:1 ↔ Minifix D15 & Dowel L34 & Cap D15 PB T18 RH:36
- Pillar Board Side Plane :35 [Flush] (18 mm): COM_02:1 ↔ Minifix D15 & Dowel L34 & Cap D15 PB T18 RH:36
- Axis Plane:52 [Mate]: COM_04:1 ↔ Minifix D15 & Dowel L34 & Cap D15 PB T18 LH:37
- Nestled Board Plane:36 [Mate]: COM_04:1 ↔ Minifix D15 & Dowel L34 & Cap D15 PB T18 LH:37
- Pillar Board Side Plane :36 [Flush] (18 mm): COM_02:1 ↔ Minifix D15 & Dowel L34 & Cap D15 PB T18 LH:37
- Axis Plane:53 [Mate]: COM_05:1 ↔ Minifix D15 & Dowel L34 & Cap D15 PB T18 RH:38
- Nestled Board Plane:37 [Mate]: COM_05:1 ↔ Minifix D15 & Dowel L34 & Cap D15 PB T18 RH:38
- Pillar Board Side Plane :37 [Flush] (18 mm): COM_03:1 ↔ Minifix D15 & Dowel L34 & Cap D15 PB T18 RH:38
- Axis Plane:54 [Mate]: COM_05:1 ↔ Minifix D15 & Dowel L34 & Cap D15 PB T18 BT:39
- Nestled Board Plane:38 [Mate]: COM_05:1 ↔ Minifix D15 & Dowel L34 & Cap D15 PB T18 BT:39
- Pillar Board Side Plane :38 [Flush] (18 mm): COM_03:1 ↔ Minifix D15 & Dowel L34 & Cap D15 PB T18 BT:39
- Axis Plane:55 [Mate]: COM_05:1 ↔ Minifix D15 & Dowel L34 & Cap D15 PB T18 LH:40
- Nestled Board Plane:39 [Mate]: COM_05:1 ↔ Minifix D15 & Dowel L34 & Cap D15 PB T18 LH:40
- Pillar Board Side Plane :39 [Flush] (18 mm): COM_03:1 ↔ Minifix D15 & Dowel L34 & Cap D15 PB T18 LH:40
- Axis Plane:56 [Mate]: COM_14:1 ↔ Minifix D15 & Dowel L34 & Cap D15 PB T18 LH:41
- Nestled Board Plane:40 [Mate]: COM_14:1 ↔ Minifix D15 & Dowel L34 & Cap D15 PB T18 LH:41
- Pillar Board Side Plane :40 [Flush] (18 mm): COM_17:1 ↔ Minifix D15 & Dowel L34 & Cap D15 PB T18 LH:41
- Axis Plane:57 [Mate]: COM_14:1 ↔ Minifix D15 & Dowel L34 & Cap D15 PB T18 BT:42
- Nestled Board Plane:41 [Mate]: COM_14:1 ↔ Minifix D15 & Dowel L34 & Cap D15 PB T18 BT:42
- Pillar Board Side Plane :41 [Flush] (18 mm): COM_17:1 ↔ Minifix D15 & Dowel L34 & Cap D15 PB T18 BT:42
- Axis Plane:58 [Mate]: COM_14:1 ↔ Minifix D15 & Dowel L34 & Cap D15 PB T18 RH:43
- Nestled Board Plane:42 [Mate]: COM_14:1 ↔ Minifix D15 & Dowel L34 & Cap D15 PB T18 RH:43
- Pillar Board Side Plane :42 [Flush] (18 mm): COM_17:1 ↔ Minifix D15 & Dowel L34 & Cap D15 PB T18 RH:43
- Axis Plane:59 [Mate]: COM_08:1 ↔ Dowel 8x30 PB T=18:1
- Nestled Board Plane:43 [Mate]: COM_25:1 ↔ Dowel 8x30 PB T=18:1
- Pillar Board Plane:1 [Mate] (-9 mm): COM_08:1 ↔ Dowel 8x30 PB T=18:1
- Axis Plane:60 [Mate]: COM_08:1 ↔ Dowel 8x30 PB T=18:2
- Nestled Board Plane:44 [Mate]: COM_25:1 ↔ Dowel 8x30 PB T=18:2
- Pillar Board Plane:2 [Mate] (-9 mm): COM_08:1 ↔ Dowel 8x30 PB T=18:2
- Axis Plane:61 [Mate]: COM_13:1 ↔ Dowel 8x30 PB T=18:3
- Nestled Board Plane:45 [Mate]: COM_25:1 ↔ Dowel 8x30 PB T=18:3
- Pillar Board Plane:3 [Mate] (-9 mm): COM_08:1 ↔ Dowel 8x30 PB T=18:3
- Axis Plane:62 [Mate]: COM_13:1 ↔ Dowel 8x30 PB T=18:4
- Nestled Board Plane:46 [Mate]: COM_25:1 ↔ Dowel 8x30 PB T=18:4
- Pillar Board Plane:4 [Mate] (-9 mm): COM_08:1 ↔ Dowel 8x30 PB T=18:4
- Axis Plane:63 [Mate]: COM_08:1 ↔ Dowel 8x30 PB T=18:5
- Nestled Board Plane:47 [Mate]: COM_04:1 ↔ Dowel 8x30 PB T=18:5
- Pillar Board Plane:5 [Mate] (-9 mm): COM_08:1 ↔ Dowel 8x30 PB T=18:5
- Axis Plane:64 [Mate]: COM_08:1 ↔ Dowel 8x30 PB T=18:6
- Nestled Board Plane:48 [Mate]: COM_04:1 ↔ Dowel 8x30 PB T=18:6
- Pillar Board Plane:6 [Mate] (-9 mm): COM_08:1 ↔ Dowel 8x30 PB T=18:6
- Axis Plane:65 [Mate]: COM_13:1 ↔ Dowel 8x30 PB T=18:7
- Nestled Board Plane:49 [Mate]: COM_25:1 ↔ Dowel 8x30 PB T=18:7
- Pillar Board Plane:7 [Mate] (-9 mm): COM_13:1 ↔ Dowel 8x30 PB T=18:7
- Axis Plane:66 [Mate]: COM_13:1 ↔ Dowel 8x30 PB T=18:8
- Nestled Board Plane:50 [Mate]: COM_25:1 ↔ Dowel 8x30 PB T=18:8
- Pillar Board Plane:8 [Mate] (-9 mm): COM_13:1 ↔ Dowel 8x30 PB T=18:8
- Axis Plane:67 [Mate]: COM_13:1 ↔ Dowel 8x30 PB T=18:9
- Nestled Board Plane:51 [Mate]: COM_24:1 ↔ Dowel 8x30 PB T=18:9
- Pillar Board Plane:9 [Mate] (-9 mm): COM_13:1 ↔ Dowel 8x30 PB T=18:9
- Axis Plane:68 [Mate]: COM_13:1 ↔ Dowel 8x30 PB T=18:10
- Nestled Board Plane:52 [Mate]: COM_24:1 ↔ Dowel 8x30 PB T=18:10
- Pillar Board Plane:10 [Mate] (-9 mm): COM_13:1 ↔ Dowel 8x30 PB T=18:10
- Flush:46 (-80 mm): COM_06:1
- Flush:47 (-80 mm): COM_06:1
- Hinge Center Axis Plane:1 [Mate]: Full Overlay Hinge Wood Screw Cup Wood Screw T18:1
- Cabinet Body Front  Edge Planar Face:1 [Mate]: COM_11:1 ↔ Full Overlay Hinge Wood Screw Cup Wood Screw T18:1
- Cabinet body Side Planar Face:1 [Flush]: COM_11:1 ↔ Full Overlay Hinge Wood Screw Cup Wood Screw T18:1
- Hinge Center Axis Plane:2 [Mate]: Full Overlay Hinge Wood Screw Cup Wood Screw T18:2
- Cabinet Body Front  Edge Planar Face:2 [Mate]: COM_11:1 ↔ Full Overlay Hinge Wood Screw Cup Wood Screw T18:2
- Cabinet body Side Planar Face:2 [Flush]: COM_11:1 ↔ Full Overlay Hinge Wood Screw Cup Wood Screw T18:2
- Axis Plane:69 [Mate]: COM_23:1 ↔ Minifix D15 & Dowel L34 & Cap D15 PB T18 LH:45
- Nestled Board Plane:53 [Mate]: COM_11:1 ↔ Minifix D15 & Dowel L34 & Cap D15 PB T18 LH:45
- Pillar Board Side Plane :43 [Flush] (18 mm): COM_02:1 ↔ Minifix D15 & Dowel L34 & Cap D15 PB T18 LH:45
- Axis Plane:70 [Mate]: COM_23:1 ↔ Minifix D15 & Dowel L34 & Cap D15 PB T18 RH:46
- Nestled Board Plane:54 [Mate]: COM_11:1 ↔ Minifix D15 & Dowel L34 & Cap D15 PB T18 RH:46
- Pillar Board Side Plane :44 [Flush] (18 mm): COM_02:1 ↔ Minifix D15 & Dowel L34 & Cap D15 PB T18 RH:46
## Named parameters: Between_Drawers = 180.5 mm, Between_Shelfs = 239.66667 mm
